# Autodesk Inventor assembly: ASM IMU
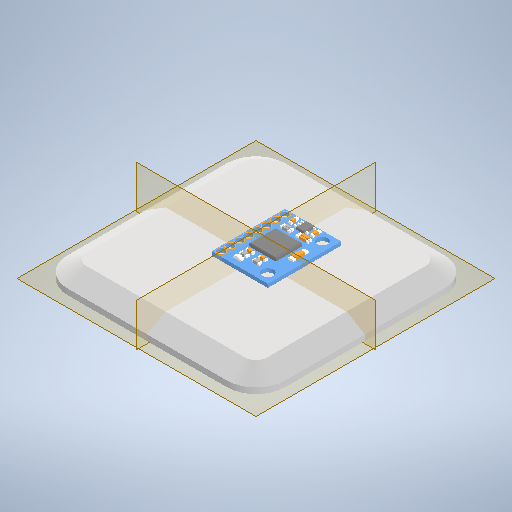
[picture p0: Inventor's stored thumbnail of the model, 512x512]
Saved by Autodesk Inventor 2025.2 (Build 292293000, 293)
## iProperties
Created: 2024-11-14
Part Number: ASM IMU
Document SubType Name: Assembly
Designer: matss
Author: matss
## Documents named in this file (3)
- C:\Users\matss\Documents\.Studium\Health Device\CAD\Wearable-Health-Device\ASM IMU.iam
- C:\Users\matss\Documents\.Studium\Health Device\CAD\Wearable-Health-Device\MPU6050 v2\MPU6050 v2\MPU6050 v2.ipt
- C:\Users\matss\Documents\.Studium\Health Device\CAD\Wearable-Health-Device\IMU_Base_T-Shirt.ipt
## Components (2 placed, 2 different names)
1. MPU6050 v2:1
2. IMU_Base_T-Shirt:1 — Mate:1, Mate:2, Mate:3, Mate:4, Angle:1
## Relationships (5: Mate 4, Angle 1)
- Mate:1: IMU_Base_T-Shirt:1
- Mate:2: IMU_Base_T-Shirt:1
- Mate:3: IMU_Base_T-Shirt:1
- Mate:4: IMU_Base_T-Shirt:1
- Angle:1 (0 deg): IMU_Base_T-Shirt:1
